# Autodesk Inventor assembly: wheel2_MIR3
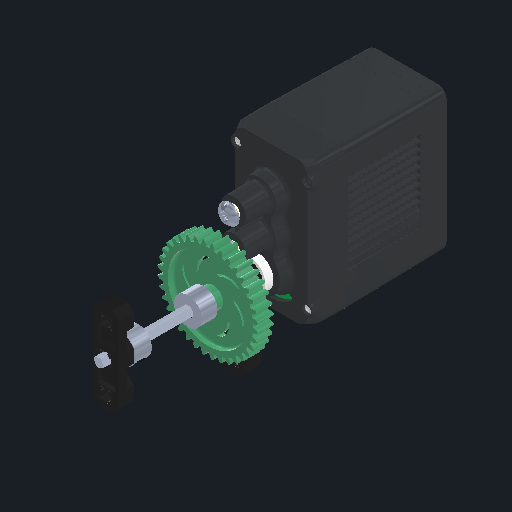
[picture p0: Inventor's stored thumbnail of the model, 512x512]
Saved by Autodesk Inventor 2024 (Build 280153000, 153)
## iProperties
Created: 2023-08-09
Part Number: wheel2_MIR3
Document SubType Name: Assembly
Designer: macbook
Author: macbook
## Documents named in this file (11)
- \\Mac\Home\Desktop\code\1899V-VRC\Cad\Assembly\v1\wheel2_MIR3.iam
- \\Mac\Home\Desktop\code\1899V-VRC\Cad\Motion\Gears\LS 36T Gear_MIR4.ipt
- \\Mac\Home\Desktop\code\1899V-VRC\Cad\Motion\Shaft LS\Shaft LS\Shaft LS 3.0.ipt
- \\Mac\Home\Desktop\code\1899V-VRC\Cad\Motion\Shaft LS\Shaft LS.ipt
- \\Mac\Home\Desktop\code\1899V-VRC\Cad\Motion\Shaft LS\Shaft Collar Metal\Shaft Collar Set Screw_MIR3.iam
- \\Mac\Home\Desktop\code\1899V-VRC\Cad\Electronics\Motors with Screws\AluM-StarS_MIR4.iam
- \\Mac\Home\Desktop\code\1899V-VRC\Cad\Motion\Spacers\Washer Teflon\TWasher .375 OD x .03125.ipt
- \\Mac\Home\Desktop\code\1899V-VRC\Cad\Motion\Spacers\Washer Teflon.ipt
- \\Mac\Home\Desktop\code\1899V-VRC\Cad\Motion\Shaft LS\Bearing Flat_MIR4.ipt
- \\Mac\Home\Desktop\code\1899V-VRC\Cad\Motion\Spacers\Spacer Nylon .500 OD\NSpacer White .500 OD x .125.ipt
- \\Mac\Home\Desktop\code\1899V-VRC\Cad\Motion\Spacers\Spacer Nylon .500 OD.ipt
## Components (9 placed, 7 different names)
1. LS 36T Gear_MIR4:1 — Insert:2, Insert:1
2. Shaft LS 3.0:1 — Mate:1, Cylindrical:2
3. Shaft Collar Set Screw_MIR3:1 [sub-assembly] — Insert:22
4. Shaft Collar Set Screw_MIR3:2 [sub-assembly] — Insert:2, Cylindrical:2
5. AluM-StarS_MIR4:1 [sub-assembly] — Mate:1, Flush:1, Insert:20
6. TWasher .375 OD x .03125:1 — Insert:17, Insert:1
7. Bearing Flat_MIR4:1 — Flush:1, Insert:19, Insert:21, Insert:17
8. NSpacer White .500 OD x .125:1 — Insert:19
9. Bearing Flat_MIR4:2 — Insert:22, Insert:21, Insert:20
## Relationships (10: Insert 7, Mate 1, Flush 1, CylindricalJoint 1)
- Insert:2: LS 36T Gear_MIR4:1 ↔ Shaft Collar Set Screw_MIR3:2
- Mate:1: Shaft LS 3.0:1 ↔ AluM-StarS_MIR4:1
- Flush:1: AluM-StarS_MIR4:1 ↔ Bearing Flat_MIR4:1
- Insert:19: Bearing Flat_MIR4:1 ↔ NSpacer White .500 OD x .125:1
- Insert:22: Shaft Collar Set Screw_MIR3:1 ↔ Bearing Flat_MIR4:2
- Insert:21 (44.45 mm): Bearing Flat_MIR4:1 ↔ Bearing Flat_MIR4:2
- Insert:20 (42.8625 mm): AluM-StarS_MIR4:1 ↔ Bearing Flat_MIR4:2
- Insert:17 (1.5875 mm): TWasher .375 OD x .03125:1 ↔ Bearing Flat_MIR4:1
- Insert:1: LS 36T Gear_MIR4:1 ↔ TWasher .375 OD x .03125:1
- Cylindrical:2: Shaft LS 3.0:1 ↔ Shaft Collar Set Screw_MIR3:2
